# Autodesk Inventor assembly: ASSEMBLY_Stack
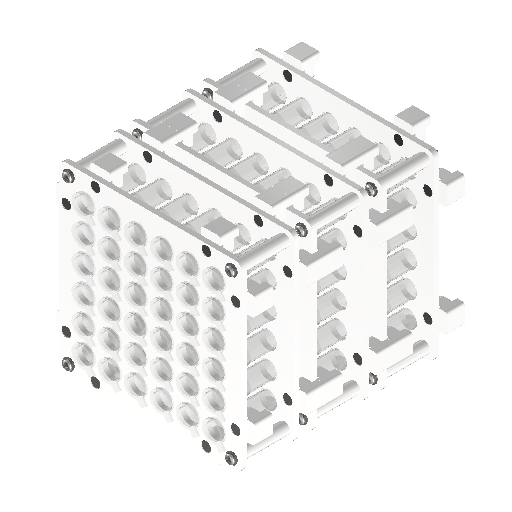
[picture p0: Inventor's stored thumbnail of the model, 512x512]
Saved by Autodesk Inventor 2026.1 (Build 301233000, 233)
## iProperties
Created: 2024-11-30
Part Number: ASSEMBLY_Stack
Document SubType Name: Assembly
Designer: User
Author: User
## Documents named in this file (2)
- C:\Users\Andrzej\OneDrive\_DRIVE_SYNCH_FILES\__ BYTECHLAB PROJECTS\MECH - SMD Parts Organizer\MCAD\1_REV1\ASSEMBLY_MAIN_REVA\ASSEMBLY_Stack.iam
- C:\Users\Andrzej\OneDrive\_DRIVE_SYNCH_FILES\__ BYTECHLAB PROJECTS\MECH - SMD Parts Organizer\MCAD\1_REV1\ASSEMBLY_MAIN_REVA\ASSEMBLY_Main.iam
## Components (3 placed, 1 different names)
1. ASSEMBLY_Main:1 [sub-assembly]
2. ASSEMBLY_Main:2 [sub-assembly]
3. ASSEMBLY_Main:3 [sub-assembly]
## Component patterns: (3 elements, first: ASSEMBLY_Main:1)
